# Autodesk Inventor assembly: Bateria
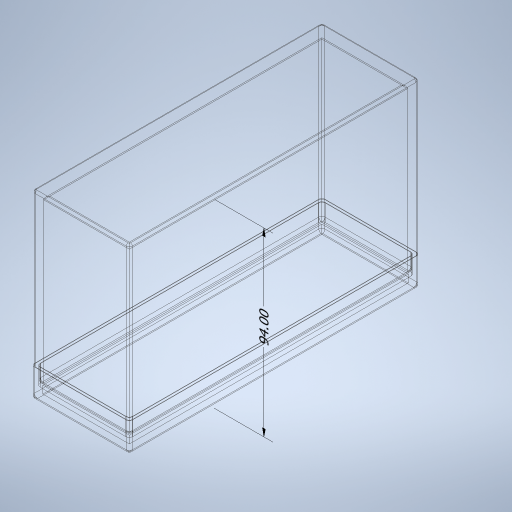
[picture p0: Inventor's stored thumbnail of the model, 512x512]
Saved by Autodesk Inventor 2024.2 (Build 282272000, 272)
## iProperties
Created: 2024-12-01
Part Number: Bateria
Document SubType Name: Assembly
Designer: sergi
Author: sergi
## Documents named in this file (3)
- C:\Users\sergi\OneDrive\Escritorio\proyectos\Moto y coche\Bateria.iam
- C:\Users\sergi\OneDrive\Escritorio\proyectos\Moto y coche\Caja bateria.ipt
- C:\Users\sergi\OneDrive\Escritorio\proyectos\Moto y coche\Tapa bateria.ipt
## Components (2 placed, 2 different names)
1. Caja bateria:1 — Nivelación:1
2. Tapa bateria:1 — Nivelación:1
## Relationships (1: Flush 1)
- Nivelación:1 [Flush]: Caja bateria:1 ↔ Tapa bateria:1
